# Autodesk Inventor assembly: StressArmAssembly
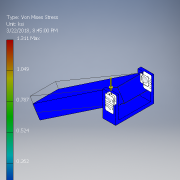
[picture p0: Inventor's stored thumbnail of the model, 180x180]
Saved by Autodesk Inventor 2017 (Build 210142000, 142)
## iProperties
Created: 2018-03-23
Part Number: StressArmAssembly
Document SubType Name: Assembly
Designer: User
Author: User
## Documents named in this file (9)
- C:\Robotics\CAD\2018-19_CAD\Offseason\StressArmAssembly.iam
- C:\Robotics\CAD\2018-19_CAD\Offseason\StressProngs.ipt
- C:\Robotics\CAD\2018-19_CAD\Offseason\StressArm.ipt
- C:\Robotics\CAD\2018-19_CAD\Offseason\StressArmAssembly\AIP\FEA\cgkfvs22o.fins
- C:\Robotics\CAD\2018-19_CAD\Offseason\StressArmAssembly\AIP\FEA\cgkfvs22o.fsat
- C:\Robotics\CAD\2018-19_CAD\Offseason\StressArmAssembly\AIP\FEA\cgkfvs22o.ftes
- C:\Robotics\CAD\2018-19_CAD\Offseason\StressArmAssembly\AIP\FEA\cgkfvs22o.fwiz
- C:\Robotics\CAD\2018-19_CAD\Offseason\StressArmAssembly\AIP\FEA\cgkfvs24g.fmsh
- C:\Robotics\CAD\2018-19_CAD\Offseason\StressArmAssembly\AIP\FEA\cgkfvs24h.fres
## Components (2 placed, 2 different names)
1. StressProngs:1 — Insert:1
2. StressArm:1 — Insert:1
## Relationships (1: Insert 1)
- Insert:1: StressProngs:1 ↔ StressArm:1
## Named parameters: sa_0 = 980.999
note: some values were not read from the file. Shown as the stored number, unit unknown: "sa_0".
